# Autodesk Inventor assembly: Big Bearing Cover Assembled
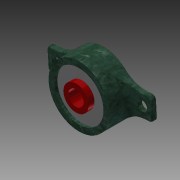
[picture p0: Inventor's stored thumbnail of the model, 180x180]
Saved by Autodesk Inventor 2014 (Build 180170000, 170)
## iProperties
Created: 2015-02-12
Part Number: Big Bearing Cover Assembled
Document SubType Name: Assembly
Designer: Spooner
Author: Spooner
## Documents named in this file (5)
- C:\Users\Spooner\Documents\Inventor\80-20  Linear Bearing\Big Bearing Cover Assembled.iam
- C:\Users\Spooner\Documents\Inventor\80-20  Linear Bearing\Big Bearing.ipt
- C:\Users\Spooner\Documents\Inventor\80-20  Linear Bearing\Big Bearing Sleeve.ipt
- C:\Users\Spooner\Documents\Inventor\80-20  Linear Bearing\Big Bearing Mount.ipt
- C:\Users\Spooner\Documents\Inventor\80-20  Linear Bearing\Big Bearing Spacer.ipt
## Components (4 placed, 4 different names)
1. Big Bearing:1 — Insert:1, Insert:2, Insert:3
2. Big Bearing Sleeve:1 — Insert:2
3. Big Bearing Mount:1 — Insert:1
4. Big Bearing Spacer:1 — Insert:3
## Relationships (3: Insert 3)
- Insert:1: Big Bearing:1 ↔ Big Bearing Mount:1
- Insert:2: Big Bearing:1 ↔ Big Bearing Sleeve:1
- Insert:3: Big Bearing:1 ↔ Big Bearing Spacer:1
